# Autodesk Inventor assembly: CycloidalGear
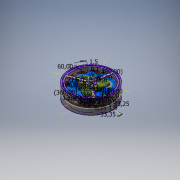
[picture p0: Inventor's stored thumbnail of the model, 180x180]
Saved by Autodesk Inventor 2018.3 (Build 223284000, 284)
## iProperties
Created: 2018-07-20
Part Number: CycloidalGear
Material: Generisch
Document SubType Name: Assembly
Designer: JochenAlt
Author: JochenAlt
## Documents named in this file (11)
- D:\Projects\FlowerPot\CAD\CycloidalGear\CycloidalGear.iam
- D:\Projects\FlowerPot\CAD\CycloidalGear\ExcentricShaft.ipt
- D:\Projects\FlowerPot\CAD\CycloidalGear\Excenter1.ipt
- D:\Projects\FlowerPot\CAD\CycloidalGear\Enclosure.ipt
- D:\Projects\FlowerPot\CAD\CycloidalGear\Rotor.ipt
- D:\Projects\FlowerPot\CAD\CycloidalGear\Excenter2.ipt
- Excenter1.ipt
- D:\Projects\FlowerPot\CAD\CycloidalGear\ExcentricMotorShaft.ipt
- D:\Projects\FlowerPot\CAD\CycloidalGear\W 61700 X-2RS1.iam
- D:\Projects\FlowerPot\CAD\CycloidalGear\ShaftHolder.ipt
- D:\Projects\FlowerPot\CAD\CycloidalGear\ShaftHolder2.ipt
## Components (18 placed, 8 different names)
1. Enclosure:1 — Passend:72, Fluchtend:24, Passend:124, Passend:125, Fluchtend:35, Fluchtend:36, Passend:129, Passend:130, Fluchtend:39, Passend:136, Passend:139, Passend:140
2. ExcentricShaft:3 — Fluchtend:23, Passend:99, Passend:104, Passend:109, Passend:133
3. Excenter1:2 — Fluchtend:23, Passend:104, Passend:108, Passend:109, Drehung:4, Drehung:5, Drehung:6, Drehung:7, Fluchtend:31, Fluchtend:32, Fluchtend:33, Passend:114, Passend:115, Passend:117, Passend:118, Passend:119, Fluchtend:34, Fluchtend:35, Drehung:10
4. Rotor:1 — Passend:131, Passend:132, Passend:133, Fluchtend:38
5. Excenter1:3 — Fluchtend:24, Passend:99, Fluchtend:25, Fluchtend:26, Passend:107, Passend:110, Drehung:2, Drehung:3, Drehung:8, Fluchtend:27, Passend:111, Fluchtend:29, Passend:112, Passend:113, Fluchtend:30, Passend:116, Fluchtend:36, Drehung:9, Fluchtend:39, Fluchtend:40
6. MotorExcentricShaft:5 — Drehung:9, Drehung:10, Passend:136, Passend:137, Passend:138, Fluchtend:40
7. ExcentricShaft:6 — Fluchtend:25, Passend:118, Passend:131
8. ExcentricShaft:7 — Fluchtend:26, Passend:107, Passend:108, Passend:132, Fluchtend:38
9. W 61700 X-2RS1:1 [sub-assembly] — Drehung:8, Passend:111, Passend:112, Passend:138
10. W 61700 X-2RS1:2 [sub-assembly] — Drehung:7, Fluchtend:32, Passend:115, Passend:137
11. W 61700 X-2RS1:3 [sub-assembly] — Passend:110, Fluchtend:29
12. W 61700 X-2RS1:4 [sub-assembly] — Drehung:6, Fluchtend:31, Passend:117
13. W 61700 X-2RS1:5 [sub-assembly] — Drehung:5, Fluchtend:33, Passend:114
14. W 61700 X-2RS1:6 [sub-assembly] — Drehung:4, Passend:119, Fluchtend:34
15. W 61700 X-2RS1:7 [sub-assembly] — Drehung:3, Passend:113, Fluchtend:30
16. W 61700 X-2RS1:8 [sub-assembly] — Drehung:2, Fluchtend:27, Passend:116
17. ShaftHolder:1 — Passend:124, Passend:125
18. ShaftHolder2:1 — Passend:129, Passend:130
## Relationships (53: Mate 28, Flush 16, RelateRotation 9)
- Passend:72 [Mate]: Enclosure:1
- Fluchtend:23 [Flush]: ExcentricShaft:3 ↔ Excenter1:2
- Fluchtend:24 [Flush]: Enclosure:1 ↔ Excenter1:3
- Passend:99 [Mate]: ExcentricShaft:3 ↔ Excenter1:3
- Passend:104 [Mate]: ExcentricShaft:3 ↔ Excenter1:2
- Fluchtend:25 [Flush]: Excenter1:3 ↔ ExcentricShaft:6
- Fluchtend:26 [Flush]: Excenter1:3 ↔ ExcentricShaft:7
- Passend:107 [Mate]: Excenter1:3 ↔ ExcentricShaft:7
- Passend:108 [Mate]: Excenter1:2 ↔ ExcentricShaft:7
- Passend:109 [Mate]: ExcentricShaft:3 ↔ Excenter1:2
- Passend:110 [Mate]: Excenter1:3 ↔ W 61700 X-2RS1:3
- Drehung:2 [RelateRotation] (1 ul): Excenter1:3 ↔ W 61700 X-2RS1:8
- Drehung:3 [RelateRotation] (1 ul): Excenter1:3 ↔ W 61700 X-2RS1:7
- Drehung:4 [RelateRotation] (1 ul): Excenter1:2 ↔ W 61700 X-2RS1:6
- Drehung:5 [RelateRotation] (1 ul): Excenter1:2 ↔ W 61700 X-2RS1:5
- Drehung:6 [RelateRotation] (1 ul): Excenter1:2 ↔ W 61700 X-2RS1:4
- Drehung:7 [RelateRotation] (1 ul): Excenter1:2 ↔ W 61700 X-2RS1:2
- Drehung:8 [RelateRotation] (1 ul): Excenter1:3 ↔ W 61700 X-2RS1:1
- Fluchtend:27 [Flush]: Excenter1:3 ↔ W 61700 X-2RS1:8
- Passend:111 [Mate]: Excenter1:3 ↔ W 61700 X-2RS1:1
- Fluchtend:29 [Flush]: Excenter1:3 ↔ W 61700 X-2RS1:3
- Passend:112 [Mate]: Excenter1:3 ↔ W 61700 X-2RS1:1
- Passend:113 [Mate]: Excenter1:3 ↔ W 61700 X-2RS1:7
- Fluchtend:30 [Flush]: Excenter1:3 ↔ W 61700 X-2RS1:7
- Fluchtend:31 [Flush]: Excenter1:2 ↔ W 61700 X-2RS1:4
- Fluchtend:32 [Flush]: Excenter1:2 ↔ W 61700 X-2RS1:2
- Fluchtend:33 [Flush]: Excenter1:2 ↔ W 61700 X-2RS1:5
- Passend:114 [Mate]: Excenter1:2 ↔ W 61700 X-2RS1:5
- Passend:115 [Mate]: Excenter1:2 ↔ W 61700 X-2RS1:2
- Passend:116 [Mate]: Excenter1:3 ↔ W 61700 X-2RS1:8
- Passend:117 [Mate]: Excenter1:2 ↔ W 61700 X-2RS1:4
- Passend:118 [Mate]: Excenter1:2 ↔ ExcentricShaft:6
- Passend:119 [Mate]: Excenter1:2 ↔ W 61700 X-2RS1:6
- Fluchtend:34 [Flush]: Excenter1:2 ↔ W 61700 X-2RS1:6
- Passend:124 [Mate]: Enclosure:1 ↔ ShaftHolder:1
- Passend:125 [Mate]: Enclosure:1 ↔ ShaftHolder:1
- Fluchtend:35 [Flush]: Enclosure:1 ↔ Excenter1:2
- Fluchtend:36 [Flush]: Enclosure:1 ↔ Excenter1:3
- Drehung:9 [RelateRotation] (-0.0909 ul): Excenter1:3 ↔ MotorExcentricShaft:5
- Drehung:10 [RelateRotation] (-0.0909 ul): Excenter1:2 ↔ MotorExcentricShaft:5
- Passend:129 [Mate]: Enclosure:1 ↔ ShaftHolder2:1
- Passend:130 [Mate]: Enclosure:1 ↔ ShaftHolder2:1
- Passend:131 [Mate]: Rotor:1 ↔ ExcentricShaft:6
- Passend:132 [Mate]: Rotor:1 ↔ ExcentricShaft:7
- Passend:133 [Mate]: ExcentricShaft:3 ↔ Rotor:1
- Fluchtend:38 [Flush]: Rotor:1 ↔ ExcentricShaft:7
- Fluchtend:39 [Flush]: Enclosure:1 ↔ Excenter1:3
- Passend:136 [Mate]: Enclosure:1 ↔ MotorExcentricShaft:5
- Passend:137 [Mate]: MotorExcentricShaft:5 ↔ W 61700 X-2RS1:2
- Passend:138 [Mate]: MotorExcentricShaft:5 ↔ W 61700 X-2RS1:1
- Fluchtend:40 [Flush]: Excenter1:3 ↔ MotorExcentricShaft:5
- Passend:139 [Mate]: Enclosure:1
- Passend:140 [Mate]: Enclosure:1
